# Autodesk Inventor assembly: Lever Arm
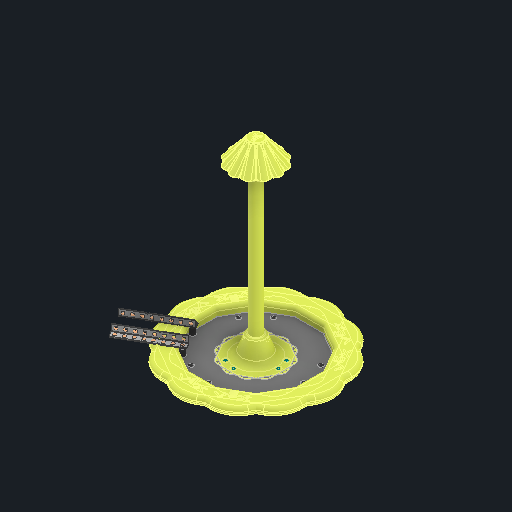
[picture p0: Inventor's stored thumbnail of the model, 512x512]
Saved by Autodesk Inventor 2025 (Build 290162000, 162)
## iProperties
Created: 2024-12-22
Part Number: Lever Arm
Document SubType Name: Assembly
Designer: Averey Ku
Author: Averey Ku
## Documents named in this file (7)
- D:\VEX\High Stakes\CAD\V4\Clamp\Lever Arm.iam
- D:\VEX\High Stakes\V5RC High Stakes Field\276-8868-200.iam
- D:\VEX\High Stakes\CAD\ROBOPROS-CAD-Inventor\Motion\Spacers\Spacer Nylon .375 OD\NSpacer .375 OD x .500.ipt
- D:\VEX\High Stakes\CAD\ROBOPROS-CAD-Inventor\Motion\Spacers\Spacer Nylon .375 OD.ipt
- D:\VEX\High Stakes\CAD\ROBOPROS-CAD-Inventor\Motion\Spacers\Washer Steel\SWasher .375 OD x .062500.ipt
- D:\VEX\High Stakes\CAD\ROBOPROS-CAD-Inventor\Motion\Spacers\Washer Steel.ipt
- D:\VEX\High Stakes\CAD\ROBOPROS-CAD-Inventor\Structure\Angle\Aluminum 1x1\Alu Angle 1x1x8.ipt
## Components (8 placed, 4 different names)
1. 276-8868-200:1 [sub-assembly] — Mate:1, Angle:1, Mate:2, Mate:3, Mate:4, Tangent:1, Tangent:4
2. 276-8868-200:2 [sub-assembly] — Mate:1, Angle:1, Mate:2, Tangent:2, Tangent:3
3. NSpacer .375 OD x .500:1 — Insert:1, Mate:3, Tangent:1, Tangent:2
4. SWasher .375 OD x .062500:1 — Insert:1, Insert:3
5. NSpacer .375 OD x .500:2 — Mate:4, Tangent:3, Tangent:4
6. SWasher .375 OD x .062500:2 — Insert:4
7. Alu Angle 1x1x8:1 — Insert:3, Mate:5
8. Alu Angle 1x1x8:2 — Insert:4, Mate:5
## Relationships (14: Mate 5, Insert 4, Tangent 4, Angle 1)
- Mate:1: 276-8868-200:1 ↔ 276-8868-200:2
- Angle:1 (30 deg): 276-8868-200:1 ↔ 276-8868-200:2
- Mate:2: 276-8868-200:1 ↔ 276-8868-200:2
- Insert:1: NSpacer .375 OD x .500:1 ↔ SWasher .375 OD x .062500:1
- [Insert]: NSpacer .375 OD x .500:2 ↔ SWasher .375 OD x .062500:2
- Mate:3: 276-8868-200:1 ↔ NSpacer .375 OD x .500:1
- Mate:4: 276-8868-200:1 ↔ NSpacer .375 OD x .500:2
- Tangent:1: 276-8868-200:1 ↔ NSpacer .375 OD x .500:1
- Tangent:2: 276-8868-200:2 ↔ NSpacer .375 OD x .500:1
- Tangent:3: 276-8868-200:2 ↔ NSpacer .375 OD x .500:2
- Tangent:4: 276-8868-200:1 ↔ NSpacer .375 OD x .500:2
- Insert:3: SWasher .375 OD x .062500:1 ↔ Alu Angle 1x1x8:1
- Insert:4: SWasher .375 OD x .062500:2 ↔ Alu Angle 1x1x8:2
- Mate:5: Alu Angle 1x1x8:1 ↔ Alu Angle 1x1x8:2
## Named parameters: d4_d3 = 0 mm
